# Autodesk Inventor assembly: Bio
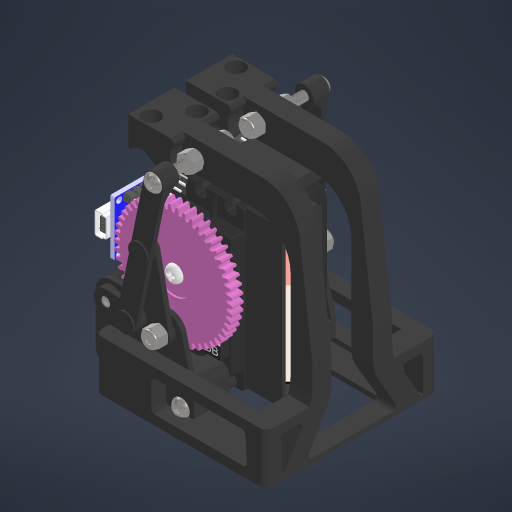
[picture p0: Inventor's stored thumbnail of the model, 512x512]
Saved by Autodesk Inventor 2024.1 (Build 281209000, 209)
## iProperties
Created: 2023-11-14
Part Number: Bio
Document SubType Name: Assembly
Designer: Brandon
Author: Brandon
## Documents named in this file (21)
- C:\Users\Brandon\Documents\School\FallCAD\Bio\Bio.iam
- C:\Users\Brandon\Documents\School\FallCAD\Bio\Servo HS425BB\Servo HS425BB.ipt
- C:\Users\Brandon\Documents\School\FallCAD\Bio\Bio\Design Accelerator\Spur Gears1.iam
- C:\Users\Brandon\Documents\School\FallCAD\Bio\Bio50t.ipt
- C:\Users\Brandon\Documents\School\FallCAD\Bio\Alignment.ipt
- C:\Users\Brandon\Documents\School\FallCAD\Bio\Bio12tNew.ipt
- C:\Users\Brandon\Documents\School\FallCAD\Bio\ServoMount.ipt
- C:\Users\Brandon\Documents\School\FallCAD\Bio\FrontLinkage.ipt
- C:\Users\Brandon\Documents\School\FallCAD\Bio\92095A179_Button Head Hex Drive Screw\92095A179_Button Head Hex Drive Screw.ipt
- C:\Users\Brandon\Documents\School\FallCAD\Bio\M3Spacer.ipt
- C:\Users\Brandon\Documents\School\FallCAD\Bio\90576A102_Medium-Strength Steel Nylon-Insert Locknut\90576A102_Medium-Strength Steel Nylon-Insert Locknut.ipt
- C:\Users\Brandon\Documents\School\FallCAD\Bio\FrontLinkage_MIR.ipt
- C:\Users\Brandon\Documents\School\FallCAD\Bio\92095A186_Button Head Hex Drive Screw\92095A186_Button Head Hex Drive Screw.ipt
- C:\Users\Brandon\Documents\School\FallCAD\Bio\Leg.ipt
- C:\Users\Brandon\Documents\School\FallCAD\Bio\Leg_MIR.ipt
- C:\Users\Brandon\Documents\School\FallCAD\Bio\91217A078_18-8 Stainless Steel Cone-Point Set Screw\91217A078_18-8 Stainless Steel Cone-Point Set Screw.ipt
- C:\Users\Brandon\Documents\School\FallCAD\Bio\AAA Battery\AAA Battery.ipt
- C:\Users\Brandon\Documents\School\FallCAD\Bio\arduino nano\arduino nano.ipt
- C:\Users\Brandon\Documents\School\FallCAD\Bio\ServoSpacer.ipt
- C:\Users\Brandon\Documents\School\FallCAD\Bio\CUI_DEVICES_TS04-66-50-BK-160-SMT\CUI_DEVICES_TS04-66-50-BK-160-SMT.iam
- C:\Users\Brandon\Documents\School\FallCAD\Bio\STLs\ElectronicsMount.ipt
## Components (32 placed, 20 different names)
1. Servo HS425BB:1 — Flush:1, Tangent:2, Mate:10
2. Bio50t:1 — Mate:1, Flush:1, Flush:2, Tangent:1
3. Alignment:1 — Mate:1, Mate:2
4. Spur Gears:1 [sub-assembly]
5. Bio12tNew:1 — Mate:2, Flush:2, Flush:3, Mate:3, Insert:1, Insert:8
6. ServoMount:1 — Insert:2, Insert:5, Insert:6, Insert:11, Insert:12, Flush:5, Mate:7, Insert:21, Insert:22, Flush:7
7. FrontLinkage:1 — Mate:3, Insert:1, Insert:3, Insert:13, Insert:15, Flush:4, Insert:19, Mate:4
8. 92095A179_Button Head Hex Drive Screw:1 — Insert:2
9. M3Spacer:1
10. 90576A102_Medium-Strength Steel Nylon-Insert Locknut:1 — Insert:3
11. 92095A179_Button Head Hex Drive Screw:3 — Insert:5
12. 90576A102_Medium-Strength Steel Nylon-Insert Locknut:2 — Insert:7
13. M3Spacer:2 — Insert:6, Insert:7
14. FrontLinkage_MIR:1 — Insert:8, Insert:14, Insert:17, Insert:20, Mate:5, Mate:6
15. 92095A186_Button Head Hex Drive Screw:1 — Insert:11
16. 92095A186_Button Head Hex Drive Screw:2 — Insert:12
17. 92095A186_Button Head Hex Drive Screw:3 — Insert:13, Insert:16, Symmetry:1
18. 92095A186_Button Head Hex Drive Screw:4 — Insert:14, Insert:18, Symmetry:1
19. Leg:1 — Flush:4, Mate:4
20. 90576A102_Medium-Strength Steel Nylon-Insert Locknut:3 — Insert:15
21. 90576A102_Medium-Strength Steel Nylon-Insert Locknut:4 — Insert:16
22. 90576A102_Medium-Strength Steel Nylon-Insert Locknut:5 — Insert:18
23. 90576A102_Medium-Strength Steel Nylon-Insert Locknut:6 — Insert:17
24. Leg_MIR:1 — Mate:5, Mate:6, Flush:6
25. 91217A078_18-8 Stainless Steel Cone-Point Set Screw:1 — Insert:20
26. 91217A078_18-8 Stainless Steel Cone-Point Set Screw:2 — Insert:19
27. AAA Battery:1 — Mate:8, Tangent:2, Flush:7
28. arduino nano:1 — Flush:5, Mate:7, Tangent:1
29. ServoSpacer:1 — Insert:21
30. ServoSpacer:2 — Insert:22
31. CUI_DEVICES_TS04-66-50-BK-160-SMT:1 [sub-assembly] — Mate:9, Mate:10
32. ElectronicsMount:1 — Flush:6
## Relationships (39: Insert 19, Mate 10, Flush 7, Tangent 2, Symmetry 1)
- Mate:1: Bio50t:1 ↔ Alignment:1
- Flush:1: Servo HS425BB:1 ↔ Bio50t:1
- Mate:2: Alignment:1 ↔ Bio12tNew:1
- Flush:2 (-0.762 mm): Bio50t:1 ↔ Bio12tNew:1
- Flush:3 (0.127 mm): Bio12tNew:1
- Mate:3: Bio12tNew:1 ↔ FrontLinkage:1
- Insert:1: Bio12tNew:1 ↔ FrontLinkage:1
- Insert:2: ServoMount:1 ↔ 92095A179_Button Head Hex Drive Screw:1
- Insert:3: FrontLinkage:1 ↔ 90576A102_Medium-Strength Steel Nylon-Insert Locknut:1
- Insert:5: ServoMount:1 ↔ 92095A179_Button Head Hex Drive Screw:3
- Insert:6: ServoMount:1 ↔ M3Spacer:2
- Insert:7: 90576A102_Medium-Strength Steel Nylon-Insert Locknut:2 ↔ M3Spacer:2
- Insert:8: Bio12tNew:1 ↔ FrontLinkage_MIR:1
- Insert:11: ServoMount:1 ↔ 92095A186_Button Head Hex Drive Screw:1
- Insert:12: ServoMount:1 ↔ 92095A186_Button Head Hex Drive Screw:2
- Insert:13: FrontLinkage:1 ↔ 92095A186_Button Head Hex Drive Screw:3
- Insert:14: FrontLinkage_MIR:1 ↔ 92095A186_Button Head Hex Drive Screw:4
- Insert:15 (5.08 mm): FrontLinkage:1 ↔ 90576A102_Medium-Strength Steel Nylon-Insert Locknut:3
- Insert:16: 92095A186_Button Head Hex Drive Screw:3 ↔ 90576A102_Medium-Strength Steel Nylon-Insert Locknut:4
- Insert:17 (5.08 mm): FrontLinkage_MIR:1 ↔ 90576A102_Medium-Strength Steel Nylon-Insert Locknut:6
- Insert:18: 92095A186_Button Head Hex Drive Screw:4 ↔ 90576A102_Medium-Strength Steel Nylon-Insert Locknut:5
- Flush:4 (9.144 mm): FrontLinkage:1 ↔ Leg:1
- Symmetry:1: 92095A186_Button Head Hex Drive Screw:3 ↔ 92095A186_Button Head Hex Drive Screw:4
- Insert:19: FrontLinkage:1 ↔ 91217A078_18-8 Stainless Steel Cone-Point Set Screw:2
- Insert:20: FrontLinkage_MIR:1 ↔ 91217A078_18-8 Stainless Steel Cone-Point Set Screw:1
- Mate:4: FrontLinkage:1 ↔ Leg:1
- Mate:5 (9.144 mm): FrontLinkage_MIR:1 ↔ Leg_MIR:1
- Mate:6: FrontLinkage_MIR:1 ↔ Leg_MIR:1
- Flush:5: ServoMount:1 ↔ arduino nano:1
- Mate:7 (2.54 mm): ServoMount:1 ↔ arduino nano:1
- Tangent:1 (0.762 mm): Bio50t:1 ↔ arduino nano:1
- Mate:8: AAA Battery:1
- Tangent:2 (1.778 mm): Servo HS425BB:1 ↔ AAA Battery:1
- Insert:21: ServoMount:1 ↔ ServoSpacer:1
- Insert:22: ServoMount:1 ↔ ServoSpacer:2
- Mate:9: CUI_DEVICES_TS04-66-50-BK-160-SMT:1
- Mate:10 (1.778 mm): Servo HS425BB:1 ↔ CUI_DEVICES_TS04-66-50-BK-160-SMT:1
- Flush:6: Leg_MIR:1 ↔ ElectronicsMount:1
- Flush:7 (4.826 mm): ServoMount:1 ↔ AAA Battery:1
